# Autodesk Inventor assembly: Custom Gears
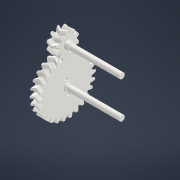
[picture p0: Inventor's stored thumbnail of the model, 180x180]
Saved by Autodesk Inventor 2022 (Build 260153000, 153)
## iProperties
Created: 2021-12-02
Part Number: Custom Gears
Document SubType Name: Assembly
Designer: izack
Author: izack
## Documents named in this file (3)
- D:\Robotics\ComputerAidedDesign\2021-22\FTC\#12456 Big Red\Drivetrain\Omni Wheel Drive\Custom Gears.iam
- D:\Robotics\ComputerAidedDesign\2021-22\FTC\#12456 Big Red\Drivetrain\Omni Wheel Drive\Shaft1.ipt
- D:\Robotics\ComputerAidedDesign\2021-22\FTC\#12456 Big Red\Drivetrain\Omni Wheel Drive\Custom Gears\Design Accelerator\Spur Gears3.iam
## Components (3 placed, 2 different names)
1. Shaft:1 — Flush:1, Mate:1, Mate:4, Mate:5
2. Shaft:2 — Flush:1, Mate:1, Mate:2, Mate:3
3. Spur Gears:1 [sub-assembly] — Mate:2, Mate:3, Mate:4, Mate:5
## Relationships (6: Mate 5, Flush 1)
- Flush:1: Shaft:1 ↔ Shaft:2
- Mate:1 (42.6466 mm): Shaft:1 ↔ Shaft:2
- Mate:2: Shaft:2 ↔ Spur Gears:1
- Mate:3: Shaft:2 ↔ Spur Gears:1
- Mate:4: Shaft:1 ↔ Spur Gears:1
- Mate:5: Shaft:1 ↔ Spur Gears:1
